# Autodesk Inventor assembly: 1.5T CAM
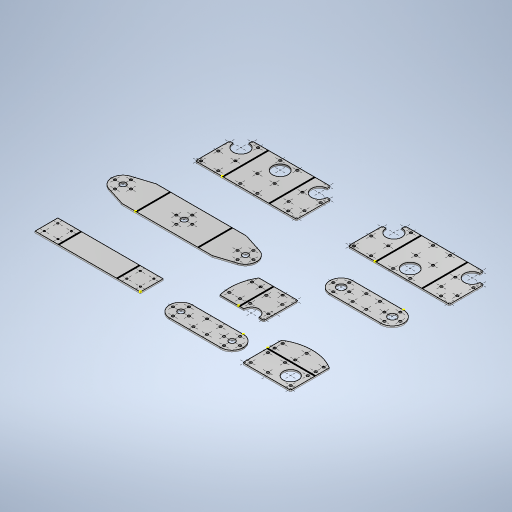
[picture p0: Inventor's stored thumbnail of the model, 512x512]
Saved by Autodesk Inventor 2024.2 (Build 282272000, 272)
## iProperties
Created: 2023-12-25
Part Number: 1.5T CAM
Document SubType Name: Assembly
Designer: chanh
Author: chanh
## Documents named in this file (9)
- C:\Users\chanh\내 드라이브\로봇\Humanoid\Roboin Humanoid Project\Inventor\rh_plus_7_axis_robot_arm_hardware\CAM\1.5T\1.5T CAM.iam
- C:\Users\chanh\내 드라이브\로봇\Humanoid\Roboin Humanoid Project\Inventor\rh_plus_7_axis_robot_arm_hardware\CAM\1.5T\Part\Flat\axis_2_bottom_L_frame(bottom).ipt
- C:\Users\chanh\내 드라이브\로봇\Humanoid\Roboin Humanoid Project\Inventor\rh_plus_7_axis_robot_arm_hardware\CAM\1.5T\Part\Flat\axis_2_bottom_L_frame(top).ipt
- C:\Users\chanh\내 드라이브\로봇\Humanoid\Roboin Humanoid Project\Inventor\rh_plus_7_axis_robot_arm_hardware\CAM\1.5T\Part\Flat\axis_3_bottom_frame(bottom).ipt
- C:\Users\chanh\내 드라이브\로봇\Humanoid\Roboin Humanoid Project\Inventor\rh_plus_7_axis_robot_arm_hardware\CAM\1.5T\Part\Flat\axis_3_bottom_frame(middle).ipt
- C:\Users\chanh\내 드라이브\로봇\Humanoid\Roboin Humanoid Project\Inventor\rh_plus_7_axis_robot_arm_hardware\CAM\1.5T\Part\Flat\axis_3_bottom_frame(top).ipt
- C:\Users\chanh\내 드라이브\로봇\Humanoid\Roboin Humanoid Project\Inventor\rh_plus_7_axis_robot_arm_hardware\CAM\1.5T\Part\Flat\axis_3_top_frame.ipt
- C:\Users\chanh\내 드라이브\로봇\Humanoid\Roboin Humanoid Project\Inventor\rh_plus_7_axis_robot_arm_hardware\CAM\1.5T\Part\Flat\axis_5_bottom_frame.ipt
- C:\Users\chanh\내 드라이브\로봇\Humanoid\Roboin Humanoid Project\Inventor\rh_plus_7_axis_robot_arm_hardware\CAM\1.5T\Part\Flat\axis_5_top_frame.ipt
## Components (8 placed, 8 different names)
1. axis_2_bottom_L_frame(bottom):1 — Mate:1, Flush:1, Mate:2
2. axis_2_bottom_L_frame(top):1 — Mate:3
3. axis_3_bottom_frame(bottom):1 — Mate:4
4. axis_3_bottom_frame(middle):1 — Mate:5
5. axis_3_bottom_frame(top):1 — Mate:6
6. axis_3_top_frame:1 — Mate:7
7. axis_5_bottom_frame:1 — Mate:8
8. axis_5_top_frame:1 — Mate:9
## Relationships (10: Mate 9, Flush 1)
- Mate:1: axis_2_bottom_L_frame(bottom):1
- Flush:1: axis_2_bottom_L_frame(bottom):1
- Mate:2: axis_2_bottom_L_frame(bottom):1
- Mate:3: axis_2_bottom_L_frame(top):1
- Mate:4: axis_3_bottom_frame(bottom):1
- Mate:5: axis_3_bottom_frame(middle):1
- Mate:6: axis_3_bottom_frame(top):1
- Mate:7: axis_3_top_frame:1
- Mate:8: axis_5_bottom_frame:1
- Mate:9: axis_5_top_frame:1
